# Autodesk Inventor assembly: Final-ass
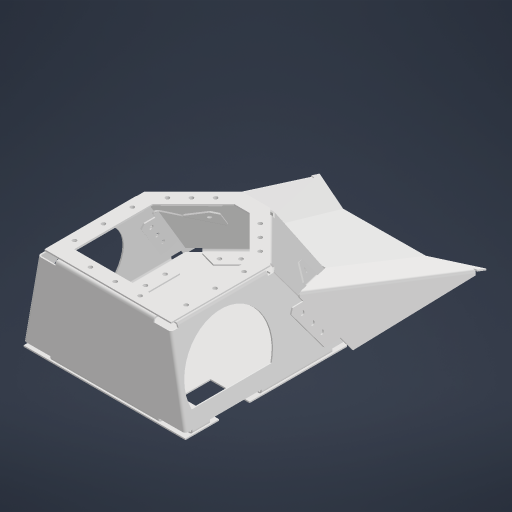
[picture p0: Inventor's stored thumbnail of the model, 512x512]
Saved by Autodesk Inventor 2023 (Build 270158000, 158)
## iProperties
Created: 2022-05-30
Part Number: Final-ass
Document SubType Name: Assembly
Designer: x43dn
Author: x43dn
## Documents named in this file (6)
- C:\Users\x43dn\Desktop\sumoltaneous-equations\sumoltaneous-equations-inventor\Final-ass.iam
- C:\Users\x43dn\Desktop\sumoltaneous-equations\sumoltaneous-equations-inventor\Bottomp.ipt
- C:\Users\x43dn\Desktop\sumoltaneous-equations\sumoltaneous-equations-inventor\Frontp.ipt
- C:\Users\x43dn\Desktop\sumoltaneous-equations\sumoltaneous-equations-inventor\Backp.ipt
- C:\Users\x43dn\Desktop\sumoltaneous-equations\sumoltaneous-equations-inventor\Topp.ipt
- C:\Users\x43dn\Desktop\sumoltaneous-equations\sumoltaneous-equations-inventor\Rampp.ipt
## Components (5 placed, 5 different names)
1. Bottomp:1 — Mate:1, Mate:2, Mate:3, Mate:4
2. Frontp:1 — Mate:1, Mate:2, Mate:7
3. Backp:1 — Mate:3, Mate:4, Mate:5, Mate:6
4. Topp:1 — Mate:5, Mate:6
5. Rampp:1 — Mate:7
## Relationships (7: Mate 7)
- Mate:1: Bottomp:1 ↔ Frontp:1
- Mate:2: Bottomp:1 ↔ Frontp:1
- Mate:3: Bottomp:1 ↔ Backp:1
- Mate:4: Bottomp:1 ↔ Backp:1
- Mate:5: Backp:1 ↔ Topp:1
- Mate:6: Backp:1 ↔ Topp:1
- Mate:7: Frontp:1 ↔ Rampp:1
